# Autodesk Inventor assembly: SolenoidRack
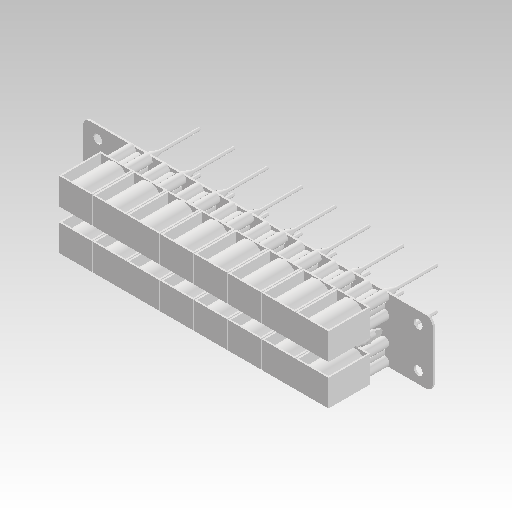
[picture p0: Inventor's stored thumbnail of the model, 512x512]
Saved by Autodesk Inventor 2020 (Build 240168000, 168)
## iProperties
Created: 2021-08-03
Part Number: SolenoidRack
Document SubType Name: Assembly
Designer: DDeGo
Author: DDeGo
## Documents named in this file (5)
- C:\Users\DDeGo\Documents\Drew\Projects\Gravity-Holo-Display\cad\SolenoidRack.iam
- C:\Users\DDeGo\Documents\Drew\Projects\Gravity-Holo-Display\cad\Solenoid.ipt
- C:\Users\DDeGo\Documents\Drew\Projects\Gravity-Holo-Display\cad\SolenoidBracket.ipt
- C:\Users\DDeGo\Documents\Drew\Projects\Gravity-Holo-Display\cad\SolenoidHead.ipt
- C:\Users\DDeGo\Documents\Drew\Projects\Gravity-Holo-Display\cad\14 Gauge Needle.ipt
## Components (49 placed, 4 different names)
1. SolenoidBracket:1 — Flush:1, Flush:2, Flush:3, Angle:1, Angle:2, Flush:4, Mate:5, Mate:6, Mate:13, Mate:14
2. 14 Gauge Needle:2 — Mate:16, Mate:17
3. 14 Gauge Needle:1 — Mate:15, Mate:18
4. SolenoidHead:2 — Mate:6, Mate:7, Mate:9, Mate:10, Mate:11, Mate:13, Mate:16, Mate:17
5. SolenoidHead:1 — Mate:5, Mate:8, Mate:9, Mate:12, Mate:14, Mate:15, Mate:18
6. Solenoid:2 — Angle:2, Mate:8, Mate:12
7. Solenoid:1 — Angle:1, Mate:7, Mate:10, Mate:11
8. 14 Gauge Needle:3
9. 14 Gauge Needle:4
10. SolenoidHead:3
11. SolenoidHead:4
12. Solenoid:3
13. Solenoid:4
14. 14 Gauge Needle:5
15. 14 Gauge Needle:6
16. SolenoidHead:5
17. SolenoidHead:6
18. Solenoid:5
19. Solenoid:6
20. 14 Gauge Needle:7
21. 14 Gauge Needle:8
22. SolenoidHead:7
23. SolenoidHead:8
24. Solenoid:7
25. Solenoid:8
26. 14 Gauge Needle:9
27. 14 Gauge Needle:10
28. SolenoidHead:9
29. SolenoidHead:10
30. Solenoid:9
31. Solenoid:10
32. 14 Gauge Needle:11
33. 14 Gauge Needle:12
34. SolenoidHead:11
35. SolenoidHead:12
36. Solenoid:11
37. Solenoid:12
38. 14 Gauge Needle:13
39. 14 Gauge Needle:14
40. SolenoidHead:13
41. SolenoidHead:14
42. Solenoid:13
43. Solenoid:14
44. 14 Gauge Needle:15
45. 14 Gauge Needle:16
46. SolenoidHead:15
47. SolenoidHead:16
48. Solenoid:15
49. Solenoid:16
## Component patterns: (8 elements, first: 14 Gauge Needle:2 + 14 Gauge Needle:1 + SolenoidHead:2 + SolenoidHead:1 + Solenoid:2 + Solenoid:1)
## Relationships (20: Mate 14, Flush 4, Angle 2)
- Flush:1: SolenoidBracket:1
- Flush:2: SolenoidBracket:1
- Flush:3: SolenoidBracket:1
- Angle:1 (0 deg): SolenoidBracket:1 ↔ Solenoid:1
- Angle:2 (0 deg): SolenoidBracket:1 ↔ Solenoid:2
- Flush:4: SolenoidBracket:1
- Mate:5: SolenoidBracket:1 ↔ SolenoidHead:1
- Mate:6: SolenoidBracket:1 ↔ SolenoidHead:2
- Mate:7: SolenoidHead:2 ↔ Solenoid:1
- Mate:8: SolenoidHead:1 ↔ Solenoid:2
- Mate:9: SolenoidHead:2 ↔ SolenoidHead:1
- Mate:10: SolenoidHead:2 ↔ Solenoid:1
- Mate:11: SolenoidHead:2 ↔ Solenoid:1
- Mate:12: SolenoidHead:1 ↔ Solenoid:2
- Mate:13: SolenoidBracket:1 ↔ SolenoidHead:2
- Mate:14: SolenoidBracket:1 ↔ SolenoidHead:1
- Mate:15: 14 Gauge Needle:1 ↔ SolenoidHead:1
- Mate:16: 14 Gauge Needle:2 ↔ SolenoidHead:2
- Mate:17: 14 Gauge Needle:2 ↔ SolenoidHead:2
- Mate:18: 14 Gauge Needle:1 ↔ SolenoidHead:1
